# Autodesk Inventor assembly: Z-powertrain(right)1
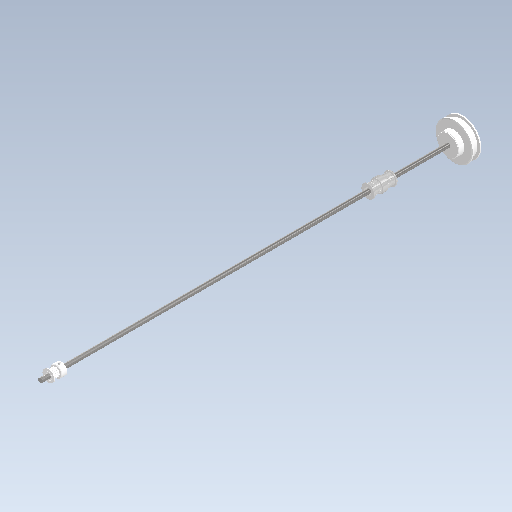
[picture p0: Inventor's stored thumbnail of the model, 512x512]
Saved by Autodesk Inventor 2020.4 (Build 244396000, 396)
## iProperties
Created: 2021-03-29
Part Number: Z-powertrain(right)1
Document SubType Name: Assembly
Designer: AOB
Mass: 34.8964 g
Surface Area: 178.662 cm^2
Volume: 30.6049 cm^3
Density: 1.14022 g/cm^3
Author: AOB
## Documents named in this file (5)
- C:\Users\marti\Documents\Inventor\ProjectBoron\Boron Ultima\Z-powertrain(right)1.iam
- C:\Users\marti\Documents\Inventor\ProjectBoron\Boron Ultima\5mm shaft(right)1.ipt
- C:\Users\marti\Documents\Inventor\ProjectBoron\Boron Ultima\GT2 16T v2 (1) (1)(right)1.ipt
- C:\Users\marti\Documents\Inventor\ProjectBoron\Boron Ultima\GT2 60T Pulley Powge(right)1.ipt
- C:\Users\marti\Documents\Inventor\ProjectBoron\Boron Ultima\double-head pulley.ipt
## Components (4 placed, 4 different names)
1. double-head pulley:1
2. 5mm shaft(right)1:1 — Flush:1, Mate:2, Flush:2, Mate:3
3. GT2 16T v2 (1) (1)(right)1:1 — Flush:1, Mate:2
4. GT2 60T Pulley Powge(right)1:1 — Flush:2, Mate:3
## Relationships (6: Mate 4, Flush 2)
- [Mate]: double-head pulley:1 ↔ 5mm shaft(right)1:1
- Flush:1 (9.5 mm): 5mm shaft(right)1:1 ↔ GT2 16T v2 (1) (1)(right)1:1
- Mate:2: 5mm shaft(right)1:1 ↔ GT2 16T v2 (1) (1)(right)1:1
- [Mate] (10 mm): double-head pulley:1 ↔ GT2 60T Pulley Powge(right)1:1
- Flush:2 (10 mm): 5mm shaft(right)1:1 ↔ GT2 60T Pulley Powge(right)1:1
- Mate:3: 5mm shaft(right)1:1 ↔ GT2 60T Pulley Powge(right)1:1
